# Autodesk Inventor assembly: Front_Frame_Fixer
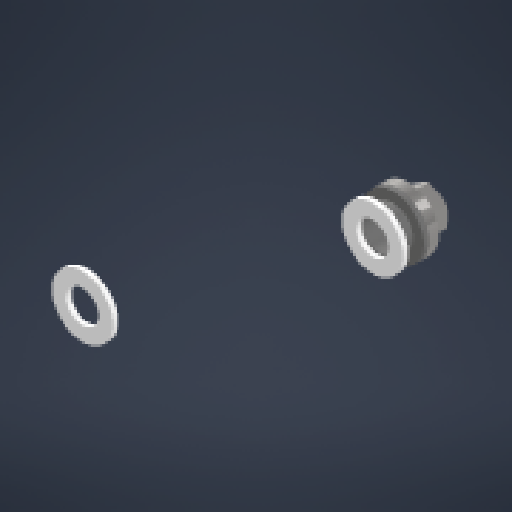
[picture p0: Inventor's stored thumbnail of the model, 512x512]
Saved by Autodesk Inventor 2024.3 (Build 283343000, 343)
## iProperties
Created: 2024-01-28
Part Number: Front_Frame_Fixer
Document SubType Name: Assembly
Designer: 김대겸
Author: 김대겸
## Documents named in this file (5)
- C:\Users\ASUS\Desktop\Anti_Backlash_Structure_OP\V2_Frame(2025)\Front_Frame_Fixer_v2.iam
- C:\Users\ASUS\Desktop\Anti_Backlash_Structure_OP\MISUMI\C-WSSA12-4-2.ipt
- C:\Users\ASUS\Desktop\Anti_Backlash_Structure_OP\MISUMI\TT-0612-10.ipt
- C:\Users\ASUS\Desktop\Anti_Backlash_Structure_OP\MISUMI\80F-0603.ipt
- C:\Users\ASUS\Desktop\Anti_Backlash_Structure_OP\MISUMI\SLBNR4.ipt
## Components (4 placed, 4 different names)
1. C-WSSA12-4-2:1
2. TT-0612-10:1
3. 80F-0603:1
4. SLBNR4:1
## Relationships (1: Insert 1)
- [Insert]: TT-0612-10:1 ↔ 80F-0603:1
